# Autodesk Inventor assembly: Assembly-Eyetracker
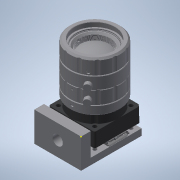
[picture p0: Inventor's stored thumbnail of the model, 180x180]
Saved by Autodesk Inventor 2022 (Build 260153000, 153)
## iProperties
Created: 2016-02-08
Part Number: Assembly-Eyetracker
Document SubType Name: Assembly
Designer: Vervaeke-Lab
Author: Vervaeke-Lab
## Documents named in this file (4)
- D:\Development\autodesk inventor models\MouseCarousel\Parts - Eyetracker\Assembly-Eyetracker.iam
- D:\Development\autodesk inventor models\MouseCarousel\Parts - Eyetracker\EdmundOptics-EO-25mm objective.ipt
- D:\Development\autodesk inventor models\MouseCarousel\Parts - Eyetracker\Workshop-BracketAdapter.ipt
- D:\Development\autodesk inventor models\MouseCarousel\Parts - Eyetracker\Basler-daA1600-60um-Basler_dart-CS-Mount_v02-Camera.ipt
## Components (3 placed, 3 different names)
1. EdmundOptics-EO-25mm objective:1 — Mate:4, Mate:5
2. Workshop-BracketAdapter:1 — Mate:1, Mate:2, Mate:3
3. Basler-daA1600-60um-Basler_dart-CS-Mount_v02-Camera:1 — Mate:1, Mate:2, Mate:3, Mate:4, Mate:5
## Relationships (5: Mate 5)
- Mate:1: Workshop-BracketAdapter:1 ↔ Basler-daA1600-60um-Basler_dart-CS-Mount_v02-Camera:1
- Mate:2: Workshop-BracketAdapter:1 ↔ Basler-daA1600-60um-Basler_dart-CS-Mount_v02-Camera:1
- Mate:3 (2.5 mm): Workshop-BracketAdapter:1 ↔ Basler-daA1600-60um-Basler_dart-CS-Mount_v02-Camera:1
- Mate:4: EdmundOptics-EO-25mm objective:1 ↔ Basler-daA1600-60um-Basler_dart-CS-Mount_v02-Camera:1
- Mate:5: EdmundOptics-EO-25mm objective:1 ↔ Basler-daA1600-60um-Basler_dart-CS-Mount_v02-Camera:1
